# Autodesk Inventor assembly: 0701 ASY GBK wall shield Center 4
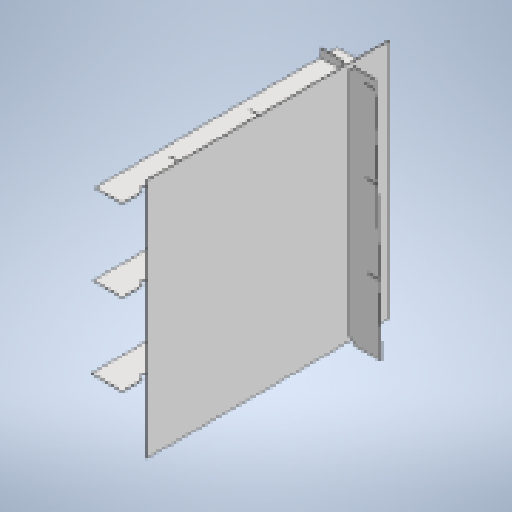
[picture p0: Inventor's stored thumbnail of the model, 512x512]
Saved by Autodesk Inventor 2026 (Build 300175000, 175)
## iProperties
Created: 2026-05-19
Part Number: 0701 ASY GBK wall shield Center 4
Document SubType Name: Assembly
Designer: pokla
Author: admin
## Documents named in this file (6)
- C:\Users\pokla\Documents\Inventor\GBK-Gubkinskiy\0701 ASY GBK wall shield Center 4.iam
- C:\Users\pokla\Documents\Inventor\GBK-Gubkinskiy\0711 GBK Center rib 2.ipt
- C:\Users\pokla\Documents\Inventor\GBK-Gubkinskiy\0713 GBK stringer C1.ipt
- C:\Users\pokla\Documents\Inventor\GBK-Gubkinskiy\05.7 GBK shield.ipt
- C:\Users\pokla\Documents\Inventor\GBK-Gubkinskiy\0714 GBK stringer C2.ipt
- C:\Users\pokla\Documents\Inventor\GBK-Gubkinskiy\0715 GBK stringer C3.ipt
## Components (6 placed, 5 different names)
1. 0711 GBK Center rib 2:1 — Заподлицо:5, Совмещение:5, Заподлицо:4, Заподлицо:6, Жесткий:1, Жесткий:2, Жесткий:3
2. 0713 GBK stringer C1:1 — Жесткий:1
3. 05.7 GBK shield:1 — Заподлицо:5, Совмещение:5, Совмещение:2, Заподлицо:1, Совмещение:1, Совмещение:4, Заподлицо:5, Заподлицо:6
4. 0711 GBK Center rib 2:2 — Заподлицо:4, Совмещение:4, Заподлицо:5
5. 0714 GBK stringer C2:1 — Жесткий:2
6. 0715 GBK stringer C3:1 — Жесткий:3
## Relationships (12: Flush 5, Mate 4, WeldJoint 3)
- Заподлицо:5 [Flush] (250 mm): 0711 GBK Center rib 2:1 ↔ 05.7 GBK shield:1
- Совмещение:5 [Mate]: 0711 GBK Center rib 2:1 ↔ 05.7 GBK shield:1
- Совмещение:2 [Mate]: 05.7 GBK shield:1
- Заподлицо:1 [Flush]: 05.7 GBK shield:1
- Совмещение:1 [Mate]: 05.7 GBK shield:1
- Заподлицо:4 [Flush]: 0711 GBK Center rib 2:1 ↔ 0711 GBK Center rib 2:2
- Совмещение:4 [Mate]: 05.7 GBK shield:1 ↔ 0711 GBK Center rib 2:2
- Заподлицо:5 [Flush]: 05.7 GBK shield:1 ↔ 0711 GBK Center rib 2:2
- Заподлицо:6 [Flush]: 0711 GBK Center rib 2:1 ↔ 05.7 GBK shield:1
- Жесткий:1 [WeldJoint] (4 mm): 0711 GBK Center rib 2:1 ↔ 0713 GBK stringer C1:1
- Жесткий:2 [WeldJoint] (4 mm): 0711 GBK Center rib 2:1 ↔ 0714 GBK stringer C2:1
- Жесткий:3 [WeldJoint] (4 mm): 0711 GBK Center rib 2:1 ↔ 0715 GBK stringer C3:1
